# Autodesk Inventor assembly: Assembly1
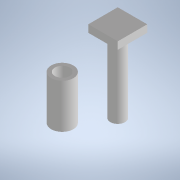
[picture p0: Inventor's stored thumbnail of the model, 180x180]
Saved by Autodesk Inventor 2022 (Build 260153000, 153)
## iProperties
Created: 2022-01-29
Part Number: Assembly1
Document SubType Name: Assembly
Designer: br4ch
Author: br4ch
## Documents named in this file (3)
- C:\Users\br4ch\M-and-Ms\HW2\Task0\Inventor\Alt\Assembly1.iam
- C:\Users\br4ch\M-and-Ms\HW2\Task0\Inventor\Alt\Shaft.ipt
- C:\Users\br4ch\M-and-Ms\HW2\Task0\Inventor\Alt\Slider.ipt
## Components (2 placed, 2 different names)
1. Shaft:1 — Mate:1
2. Slider:1 — Mate:1
## Relationships (1: Mate 1)
- Mate:1: Shaft:1 ↔ Slider:1
